# Autodesk Inventor assembly: Assembly1
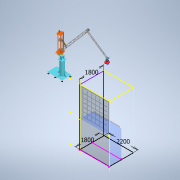
[picture p0: Inventor's stored thumbnail of the model, 180x180]
Saved by Autodesk Inventor 2020 (Build 240168000, 168)
## iProperties
Created: 2020-07-25
Part Number: Assembly1
Document SubType Name: Assembly
Designer: Vikki
Mass: 83498.3 g
Surface Area: 288732 cm^2
Volume: 3.615e+06 cm^3
Density: 0.0230977 g/cm^3
Author: Vikki
## Documents named in this file (29)
- D:\projects\Intelligent Picking\vicky models\manufacturing model-1\manufactruning model-1.iam
- D:\projects\Intelligent Picking\vicky models\manufacturing model-1\link-1 (2by1 inch ms sq tube).ipt
- D:\projects\Intelligent Picking\vicky models\manufacturing model-1\base plate.ipt
- D:\projects\Intelligent Picking\vicky models\manufacturing model-1\ms truss - 2.ipt
- D:\projects\Intelligent Picking\vicky models\manufacturing model-1\ms truss for link 3.ipt
- D:\projects\Intelligent Picking\vicky models\manufacturing model-1\manufacturing link-4.ipt
- D:\projects\Intelligent Picking\vicky models\manufacturing model-1\motor assembly (mega troque).iam
- D:\projects\Intelligent Picking\vicky models\manufacturing model-1\base for ball scew -bolt.ipt
- D:\projects\Intelligent Picking\vicky models\manufacturing model-1\connecting rod.ipt
- D:\projects\Intelligent Picking\vicky models\manufacturing model-1\endeffector motor assembly.iam
- D:\projects\Intelligent Picking\vicky models\manufacturing model-1\ball screw end thrust bearing.ipt
- D:\projects\Intelligent Picking\vicky models\manufacturing model-1\ballscrew radial ball bearing.ipt
- D:\projects\Intelligent Picking\workspace2.ipt
- D:\projects\Intelligent Picking\vicky models\manufacturing model-1\universal end effector.ipt
- D:\projects\Intelligent Picking\vicky models\manufacturing model-1\nmrv gear boxes\nmrv-50\wrom gearbox nmrv 50.iam
- D:\projects\Intelligent Picking\vicky models\manufacturing model-1\nmrv gear boxes\nmrv-40\worm gearbox nmrv 40.iam
- D:\projects\Intelligent Picking\vicky models\manufacturing model-1\nmvr-40 coupler.ipt
- D:\projects\Intelligent Picking\vicky models\manufacturing model-1\nmrv 50 0p shaft- pin.ipt
- D:\projects\Intelligent Picking\vicky models\manufacturing model-1\nmrv-50 to mega torque mototr coupler.ipt
- D:\projects\Intelligent Picking\vicky models\manufacturing model-1\nmrv-50 to megatroque motor coupler.ipt
- D:\projects\Intelligent Picking\vicky models\manufacturing model-1\ball screw astro.ipt
- D:\projects\Intelligent Picking\vicky models\manufacturing model-1\mega troque motor to nmrv-50 flange.ipt
- D:\projects\Intelligent Picking\vicky models\manufacturing model-1\mega troque motor flange for nmrv-40.ipt
- D:\projects\Intelligent Picking\vicky models\manufacturing model-1\manufactruning model-1\AIP\FEA\dbbgnjsio.fins
- D:\projects\Intelligent Picking\vicky models\manufacturing model-1\manufactruning model-1\AIP\FEA\dbbgnjsio.fsat
- D:\projects\Intelligent Picking\vicky models\manufacturing model-1\manufactruning model-1\AIP\FEA\dbbgnjsio.ftes
- D:\projects\Intelligent Picking\vicky models\manufacturing model-1\manufactruning model-1\AIP\FEA\dbbgnjsio.fwiz
- D:\projects\Intelligent Picking\vicky models\manufacturing model-1\manufactruning model-1\AIP\FEA\dbbgnjsjk.fmsh
- D:\projects\Intelligent Picking\vicky models\manufacturing model-1\manufactruning model-1\AIP\FEA\dbf3w2ops.fmsh
## Components (27 placed, 22 different names)
1. link-1 (2by1 inch ms sq tube):1 — Mate:1, Flush:8, Mate:12, Mate:13, Mate:14, Mate:15, Mate:16, Mate:17, Mate:23, Flush:18, Flush:19, Mate:36, Angle:3, Angle:12, Mate:59, Mate:61, Mate:63
2. base plate:2 — Mate:1, Mate:23, Mate:37, Angle:4, Mate:38, Mate:43, Mate:44, Angle:8, Angle:9
3. ms truss - 2:1 — Flush:8, Mate:5, Mate:14, Mate:20, Flush:15, Mate:29, Flush:16, Mate:42, Angle:7, Mate:51, Angle:13
4. ms truss for link 3:1 — Mate:5, Mate:9, Mate:25, Mate:26, Mate:27, Mate:41, Mate:51, Flush:21, Mate:54, Mate:55, Mate:56, Mate:57
5. manufacturing link-4:1 — Mate:9, Mate:28, Angle:5, Mate:39, Mate:40, Angle:6
6. motor assembly (mega troque):1 [sub-assembly] — Mate:12, Mate:13, Mate:17, Mate:64
7. base for ball scew -bolt:2 — Mate:15, Mate:16, Mate:21, Mate:58
8. connecting rod:1 — Mate:20, Mate:21, Flush:15, Mate:30
9. connecting rod:2 — Mate:29, Flush:16, Mate:30
10. endeffector motor assembly:1 [sub-assembly] — Mate:25, Mate:26, Mate:27, Mate:28
11. ball screw end thrust bearing:2 — Mate:62, Mate:63
12. ballscrew radial ball bearing:1 — Flush:18, Flush:19, Mate:61
13. workspace2:1 — Mate:36, Angle:3, Mate:37, Angle:4, Mate:38, Angle:5, Flush:30
14. universal end effector:1 — Mate:39, Mate:40, Angle:6, Flush:30
15. wrom gearbox nmrv 50:1 [sub-assembly] — Mate:41, Mate:42, Angle:7, Mate:47, Mate:48, Angle:10, Flush:21, Mate:52, Mate:53, Flush:26, Flush:27, Mate:65, Mate:67, Mate:69
16. worm gearbox nmrv 40:1 [sub-assembly] — Mate:43, Mate:44, Angle:8, Mate:45, Mate:46, Angle:11, Mate:49, Mate:50, Flush:20, Flush:23, Mate:70, Flush:28, Flush:29, Mate:72
17. motor assembly (mega troque):2 [sub-assembly] — Mate:45, Angle:9, Mate:46, Angle:11, Flush:25, Mate:71
18. motor assembly (mega troque):3 [sub-assembly] — Mate:47, Mate:48, Angle:10, Angle:13
19. nmvr-40 coupler:1 — Mate:49, Mate:50, Flush:20, Angle:12
20. nmrv 50 0p shaft- pin:1 — Mate:52, Mate:53, Mate:54
21. nmrv 50 0p shaft- pin:2 — Mate:55, Mate:56, Mate:57
22. nmrv-50 to megatroque motor coupler:1 — Flush:23, Flush:25, Mate:70
23. ball screw astro:1 — Mate:58, Mate:59, Mate:60, Mate:62
24. nmrv-50 to mega torque mototr coupler:2 — Mate:60, Mate:64
25. mega troque motor to nmrv-50 flange:1 — Flush:26, Flush:27, Mate:66, Mate:68, Mate:69
26. nmrv-50 to mega torque mototr coupler:3 — Mate:65, Mate:66, Mate:67, Mate:68
27. mega troque motor flange for nmrv-40:1 — Flush:28, Flush:29, Mate:71, Mate:72
## Relationships (80: Mate 55, Flush 14, Angle 11)
- Mate:1 (25 mm): link-1 (2by1 inch ms sq tube):1 ↔ base plate:2
- Flush:8: link-1 (2by1 inch ms sq tube):1 ↔ ms truss - 2:1
- Mate:5 (10 mm): ms truss - 2:1 ↔ ms truss for link 3:1
- Mate:9 (10 mm): ms truss for link 3:1 ↔ manufacturing link-4:1
- Mate:12: link-1 (2by1 inch ms sq tube):1 ↔ motor assembly (mega troque):1
- Mate:13: link-1 (2by1 inch ms sq tube):1 ↔ motor assembly (mega troque):1
- Mate:14: link-1 (2by1 inch ms sq tube):1 ↔ ms truss - 2:1
- Mate:15: link-1 (2by1 inch ms sq tube):1 ↔ base for ball scew -bolt:2
- Mate:16: link-1 (2by1 inch ms sq tube):1 ↔ base for ball scew -bolt:2
- Mate:17: link-1 (2by1 inch ms sq tube):1 ↔ motor assembly (mega troque):1
- Mate:20: ms truss - 2:1 ↔ connecting rod:1
- Mate:21: base for ball scew -bolt:2 ↔ connecting rod:1
- Mate:23: link-1 (2by1 inch ms sq tube):1 ↔ base plate:2
- Mate:25: ms truss for link 3:1 ↔ endeffector motor assembly:1
- Mate:26: ms truss for link 3:1 ↔ endeffector motor assembly:1
- Mate:27: ms truss for link 3:1 ↔ endeffector motor assembly:1
- Mate:28: manufacturing link-4:1 ↔ endeffector motor assembly:1
- Flush:15: ms truss - 2:1 ↔ connecting rod:1
- Mate:29: ms truss - 2:1 ↔ connecting rod:2
- Flush:16: ms truss - 2:1 ↔ connecting rod:2
- Mate:30: connecting rod:1 ↔ connecting rod:2
- Flush:18: link-1 (2by1 inch ms sq tube):1 ↔ ballscrew radial ball bearing:1
- Flush:19: link-1 (2by1 inch ms sq tube):1 ↔ ballscrew radial ball bearing:1
- Mate:36 (-1700 mm): link-1 (2by1 inch ms sq tube):1 ↔ workspace2:1
- Angle:3 (0 deg): link-1 (2by1 inch ms sq tube):1 ↔ workspace2:1
- Mate:37: base plate:2 ↔ workspace2:1
- Angle:4 (0 deg): base plate:2 ↔ workspace2:1
- Mate:38 (-500 mm): base plate:2 ↔ workspace2:1
- Angle:5 (0 deg): manufacturing link-4:1 ↔ workspace2:1
- Mate:39: manufacturing link-4:1 ↔ universal end effector:1
- Mate:40: manufacturing link-4:1 ↔ universal end effector:1
- Angle:6 (0 deg): manufacturing link-4:1 ↔ universal end effector:1
- Mate:41: ms truss for link 3:1 ↔ wrom gearbox nmrv 50:1
- Mate:42: ms truss - 2:1 ↔ wrom gearbox nmrv 50:1
- Angle:7 (0 deg): ms truss - 2:1 ↔ wrom gearbox nmrv 50:1
- Mate:43: base plate:2 ↔ worm gearbox nmrv 40:1
- Mate:44: base plate:2 ↔ worm gearbox nmrv 40:1
- Angle:8 (0 deg): base plate:2 ↔ worm gearbox nmrv 40:1
- Mate:45: worm gearbox nmrv 40:1 ↔ motor assembly (mega troque):2
- Angle:9 (90 deg): base plate:2 ↔ motor assembly (mega troque):2
- Mate:46 (10 mm): worm gearbox nmrv 40:1 ↔ motor assembly (mega troque):2
- Mate:47: wrom gearbox nmrv 50:1 ↔ motor assembly (mega troque):3
- Mate:48 (10 mm): wrom gearbox nmrv 50:1 ↔ motor assembly (mega troque):3
- Angle:10 (0 deg): wrom gearbox nmrv 50:1 ↔ motor assembly (mega troque):3
- Angle:11 (0 deg): worm gearbox nmrv 40:1 ↔ motor assembly (mega troque):2
- Mate:49: worm gearbox nmrv 40:1 ↔ nmvr-40 coupler:1
- Mate:50: worm gearbox nmrv 40:1 ↔ nmvr-40 coupler:1
- Flush:20 (-2 mm): worm gearbox nmrv 40:1 ↔ nmvr-40 coupler:1
- Angle:12 (0 deg): link-1 (2by1 inch ms sq tube):1 ↔ nmvr-40 coupler:1
- Mate:51: ms truss - 2:1 ↔ ms truss for link 3:1
- Flush:21: ms truss for link 3:1 ↔ wrom gearbox nmrv 50:1
- Angle:13 (0 deg): ms truss - 2:1 ↔ motor assembly (mega troque):3
- Mate:52: wrom gearbox nmrv 50:1 ↔ nmrv 50 0p shaft- pin:1
- Mate:53: wrom gearbox nmrv 50:1 ↔ nmrv 50 0p shaft- pin:1
- Mate:54 (-10 mm): ms truss for link 3:1 ↔ nmrv 50 0p shaft- pin:1
- Mate:55: ms truss for link 3:1 ↔ nmrv 50 0p shaft- pin:2
- Mate:56: ms truss for link 3:1 ↔ nmrv 50 0p shaft- pin:2
- Mate:57 (-12 mm): ms truss for link 3:1 ↔ nmrv 50 0p shaft- pin:2
- Flush:23: worm gearbox nmrv 40:1 ↔ nmrv-50 to megatroque motor coupler:1
- Flush:25: motor assembly (mega troque):2 ↔ nmrv-50 to megatroque motor coupler:1
- Mate:58: base for ball scew -bolt:2 ↔ ball screw astro:1
- Mate:59: link-1 (2by1 inch ms sq tube):1 ↔ ball screw astro:1
- Mate:60: ball screw astro:1 ↔ nmrv-50 to mega torque mototr coupler:2
- Mate:61: link-1 (2by1 inch ms sq tube):1 ↔ ballscrew radial ball bearing:1
- Flush:26: wrom gearbox nmrv 50:1 ↔ mega troque motor to nmrv-50 flange:1
- Flush:27: wrom gearbox nmrv 50:1 ↔ mega troque motor to nmrv-50 flange:1
- Mate:62: ball screw end thrust bearing:2 ↔ ball screw astro:1
- Mate:63: link-1 (2by1 inch ms sq tube):1 ↔ ball screw end thrust bearing:2
- Mate:64 (2 mm): motor assembly (mega troque):1 ↔ nmrv-50 to mega torque mototr coupler:2
- Mate:65: wrom gearbox nmrv 50:1 ↔ nmrv-50 to mega torque mototr coupler:3
- Mate:66 (15 mm): mega troque motor to nmrv-50 flange:1 ↔ nmrv-50 to mega torque mototr coupler:3
- Mate:67: wrom gearbox nmrv 50:1 ↔ nmrv-50 to mega torque mototr coupler:3
- Mate:68: mega troque motor to nmrv-50 flange:1 ↔ nmrv-50 to mega torque mototr coupler:3
- Mate:69: wrom gearbox nmrv 50:1 ↔ mega troque motor to nmrv-50 flange:1
- Mate:70: worm gearbox nmrv 40:1 ↔ nmrv-50 to megatroque motor coupler:1
- Flush:28: worm gearbox nmrv 40:1 ↔ mega troque motor flange for nmrv-40:1
- Flush:29: worm gearbox nmrv 40:1 ↔ mega troque motor flange for nmrv-40:1
- Mate:71: motor assembly (mega troque):2 ↔ mega troque motor flange for nmrv-40:1
- Mate:72: worm gearbox nmrv 40:1 ↔ mega troque motor flange for nmrv-40:1
- Flush:30 (120 mm): workspace2:1 ↔ universal end effector:1
## Named parameters: sa_0 = 981, sa_1 = 5000
note: some values were not read from the file. Shown as the stored number, unit unknown: "sa_0", "sa_1".
